# Autodesk Inventor assembly: 2DoF Manipulator Type 1
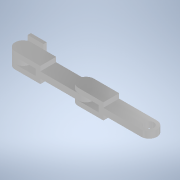
[picture p0: Inventor's stored thumbnail of the model, 180x180]
Saved by Autodesk Inventor 2021 (Build 250183000, 183)
## iProperties
Created: 2023-06-26
Part Number: 2DoF Manipulator Type 1
Document SubType Name: Assembly
Designer: fist5
Mass: 1832.42 g
Surface Area: 1155.25 cm^2
Volume: 678.673 cm^3
Density: 2.7 g/cm^3
Sending System: Autodesk Inventor 2023
Preprocessor: ST-DEVELOPER v19.2
Title: 2DoF Manipulator Type 1.stp
Author: fist5
## Documents named in this file (3)
- C:\Users\fist5\GIT LocalFiles\DGIST-MECH401-RobotDynamics\Part8_Computed Torque Control (Position Control)\Motor PID based Position Control\2DoF Manipulator Control\2DoF Manipulator Design\2DoF Manipulator Type 1.iam
- C:\Users\fist5\GIT LocalFiles\DGIST-MECH401-RobotDynamics\Part8_Computed Torque Control (Position Control)\Motor PID based Position Control\2DoF Manipulator Control\2DoF Manipulator Design\Manipulator Base Type1.ipt
- C:\Users\fist5\GIT LocalFiles\DGIST-MECH401-RobotDynamics\Part8_Computed Torque Control (Position Control)\Motor PID based Position Control\2DoF Manipulator Control\2DoF Manipulator Design\Manipulator Link Type 1.ipt
## Components (3 placed, 2 different names)
1. Manipulator Base Type1:1 — Mate:5, Mate:6
2. Manipulator Link Type 1:1 — Mate:3, Mate:4, Mate:5, Mate:6
3. Manipulator Link Type 1:2 — Mate:3, Mate:4
## Relationships (4: Mate 4)
- Mate:3: Manipulator Link Type 1:1 ↔ Manipulator Link Type 1:2
- Mate:4: Manipulator Link Type 1:1 ↔ Manipulator Link Type 1:2
- Mate:5: Manipulator Base Type1:1 ↔ Manipulator Link Type 1:1
- Mate:6: Manipulator Base Type1:1 ↔ Manipulator Link Type 1:1
